# Autodesk Inventor assembly: CAM2
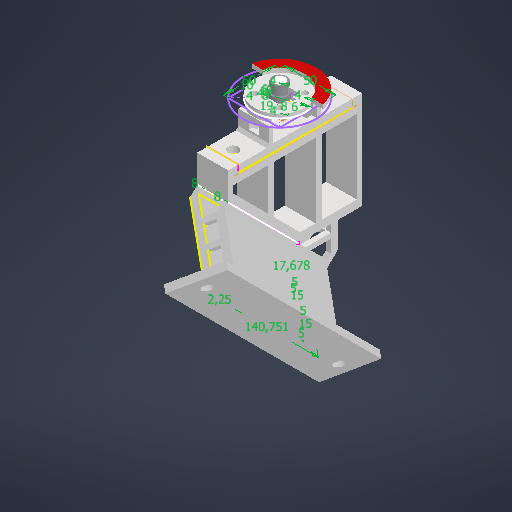
[picture p0: Inventor's stored thumbnail of the model, 512x512]
Saved by Autodesk Inventor 2026.2 (Build 302298000, 298)
## iProperties
Created: 2025-12-02
Part Number: CAM2
Document SubType Name: Assembly
Designer: alexa
Author: alexa
## Documents named in this file (4)
- E:\work\Diplomarbeit\Bauteile\CAM2.iam
- E:\work\Diplomarbeit\FIT0892\FIT0892\FIT0892.iam
- E:\work\Diplomarbeit\CAM\CAM1.ipt
- E:\work\Diplomarbeit\Bauteile\HalterungIso.ipt
## Components (3 placed, 3 different names)
1. FIT0892:1 [sub-assembly] — Fluchtend:5
2. CAM1:1 — Fluchtend:4, Fluchtend:5, Fluchtend:6, Fluchtend:7, Fluchtend:8, Fluchtend:9
3. HalterungIso:1 — Fluchtend:6, Fluchtend:7, Fluchtend:8, Fluchtend:9
## Relationships (7: Flush 7)
- Fluchtend:3 [Flush] (-5 mm)
- Fluchtend:4 [Flush]: CAM1:1
- Fluchtend:5 [Flush]: FIT0892:1 ↔ CAM1:1
- Fluchtend:6 [Flush]: CAM1:1 ↔ HalterungIso:1
- Fluchtend:7 [Flush]: CAM1:1 ↔ HalterungIso:1
- Fluchtend:8 [Flush]: CAM1:1 ↔ HalterungIso:1
- Fluchtend:9 [Flush]: CAM1:1 ↔ HalterungIso:1
## Named parameters: Finish1_Area = 8.55976
note: some values were not read from the file. Shown as the stored number, unit unknown: "Finish1_Area".
